# Autodesk Inventor assembly: Plate_link
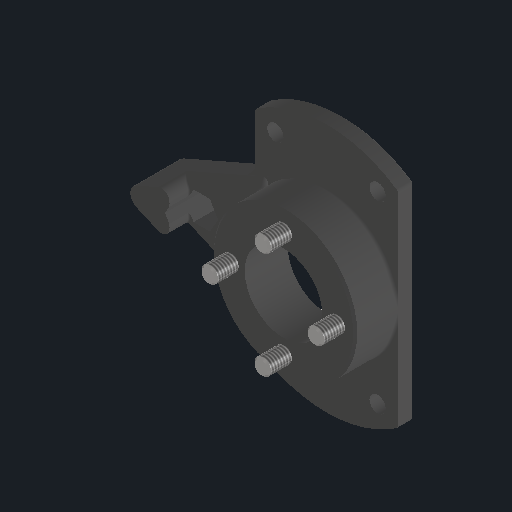
[picture p0: Inventor's stored thumbnail of the model, 512x512]
Saved by Autodesk Inventor 2022 (Build 260153070, 153G)
## iProperties
Created: 2021-11-24
Part Number: Plate_link
Document SubType Name: Assembly
Designer: Teo
Title: Predstavitev sklopa
Author: Teo
## Documents named in this file (3)
- D:\Zaključna\Roka\Priloge\IPT_files\Assemblies\Plate_link.iam
- D:\Zaključna\Roka\Priloge\IPT_files\Final_rotary_plate.ipt
- C:\Users\Teo\Documents\Inventor\Content Center Files\R2022\en-US\DIN 912\DIN 912 - M4 x 0.7 x 16 x 14.25.ipt
## Components (5 placed, 2 different names)
1. Final_rotary_plate:1 — Mate:1, Mate:2, Mate:3, Mate:4, Mate:5, Mate:6, Mate:7, Mate:8
2. DIN 912 - replaced by DIN EN ISO 4762 M4 x 16:3 — Mate:1, Mate:2
3. DIN 912 - replaced by DIN EN ISO 4762 M4 x 16:1 — Mate:3, Mate:4
4. DIN 912 - replaced by DIN EN ISO 4762 M4 x 16:2 — Mate:5, Mate:6
5. DIN 912 - replaced by DIN EN ISO 4762 M4 x 16:4 — Mate:7, Mate:8
## Relationships (8: Mate 8)
- Mate:1: Final_rotary_plate:1 ↔ DIN 912 - replaced by DIN EN ISO 4762 M4 x 16:3
- Mate:2: Final_rotary_plate:1 ↔ DIN 912 - replaced by DIN EN ISO 4762 M4 x 16:3
- Mate:3: Final_rotary_plate:1 ↔ DIN 912 - replaced by DIN EN ISO 4762 M4 x 16:1
- Mate:4: Final_rotary_plate:1 ↔ DIN 912 - replaced by DIN EN ISO 4762 M4 x 16:1
- Mate:5: Final_rotary_plate:1 ↔ DIN 912 - replaced by DIN EN ISO 4762 M4 x 16:2
- Mate:6: Final_rotary_plate:1 ↔ DIN 912 - replaced by DIN EN ISO 4762 M4 x 16:2
- Mate:7: Final_rotary_plate:1 ↔ DIN 912 - replaced by DIN EN ISO 4762 M4 x 16:4
- Mate:8: Final_rotary_plate:1 ↔ DIN 912 - replaced by DIN EN ISO 4762 M4 x 16:4
